# Autodesk Inventor assembly: HbIndexFingerForChild
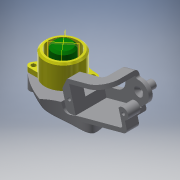
[picture p0: Inventor's stored thumbnail of the model, 180x180]
Saved by Autodesk Inventor 2017 (Build 210142000, 142)
## iProperties
Part Number: HbIndexFingerForChild
Material: 一般
Document SubType Name: Assembly
Designer: sktom
Author: sktom
## Documents named in this file (4)
- D:\OneDrive\CAD\hackberry\HACKberry-hardware\3D_69%\Hand\IndexFinger\HbIndexFingerForChild.iam
- D:\OneDrive\CAD\hackberry\HACKberry-hardware\3D_69%\Hand\ThumbFinger\HbThumbMetacarpalPhalanx02ForChild.ipt
- D:\OneDrive\CAD\hackberry\HACKberry-hardware\3D_69%\Hand\ThumbFinger\HbThumbLockButton01ForChild.ipt
- D:\OneDrive\CAD\hackberry\HACKberry-hardware\3D_69%\Hand\ThumbFinger\HbThumbJointHolder01ForChild.ipt
## Components (3 placed, 3 different names)
1. HbThumbMetacarpalPhalanx02ForChild:1 — 挿入:1, 挿入:2, 挿入:3
2. HbThumbLockButton01ForChild:1 — 挿入:3
3. HbThumbJointHolder01ForChild:1 — 挿入:1, 挿入:2
## Relationships (3: Insert 3)
- 挿入:1 [Insert]: HbThumbMetacarpalPhalanx02ForChild:1 ↔ HbThumbJointHolder01ForChild:1
- 挿入:2 [Insert]: HbThumbMetacarpalPhalanx02ForChild:1 ↔ HbThumbJointHolder01ForChild:1
- 挿入:3 [Insert] (2 mm): HbThumbMetacarpalPhalanx02ForChild:1 ↔ HbThumbLockButton01ForChild:1
